# Autodesk Inventor assembly: Tool_Revo
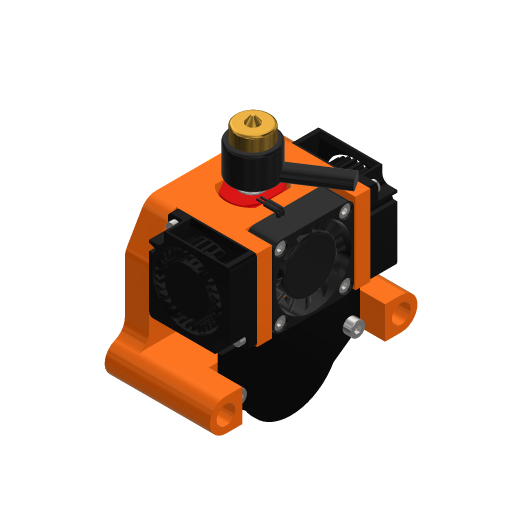
[picture p0: Inventor's stored thumbnail of the model, 512x512]
Saved by Autodesk Inventor 2023.2 (Build 272271000, 271)
## iProperties
Created: 2023-02-09
Part Number: Tool_Revo
Document SubType Name: Assembly
Designer: remop
Author: remop
## Documents named in this file (12)
- C:\Users\remop\OneDrive\Documents\Inventor\3D Printers\LuEVO\Mk5_FullKinematic\Extruders and Tools\Revo Tool\Tool_Revo.iam
- C:\Users\remop\OneDrive\Documents\Inventor\3D Printers\LuEVO\Mk5_FullKinematic\Extruders and Tools\Revo Tool\Tool_Revo.ipt
- C:\Users\remop\OneDrive\Documents\Inventor\3D Printers\LuEVO\Mk5_FullKinematic\XY Motion System\Toolhead\MagToolChanger_CouplerL.ipt
- C:\Users\remop\OneDrive\Documents\Inventor\3D Printers\LuEVO\Mk5_FullKinematic\XY Motion System\Toolhead\MagToolChanger_Magnet.ipt
- C:\Users\remop\OneDrive\Documents\Inventor\3D Printers\LuEVO\Mk5_FullKinematic\Electronics\Mellow Fly SHT36.ipt
- C:\Users\remop\OneDrive\Documents\Inventor\3D Printers\LuEVO\Mk5_FullKinematic\Extruders and Tools\Revo Tool\3010 Blower.ipt
- C:\Users\remop\OneDrive\Documents\Inventor\3D Printers\LuEVO\Mk5_FullKinematic\Extruders and Tools\Revo Tool\3010 Fan.ipt
- C:\Users\remop\OneDrive\Documents\Inventor\3D Printers\LuEVO\Mk5_FullKinematic\Extruders and Tools\Revo Tool\Revo Voron Reference CAD.ipt
- C:\Users\remop\OneDrive\Documents\Inventor\Content Center Files\R2023\en-US\BS EN ISO 4762\BS EN ISO 4762 - M2.5 x 12(1).ipt
- C:\Users\remop\OneDrive\Documents\Inventor\Content Center Files\R2023\en-US\BS EN ISO 4762\BS EN ISO 4762 - M3 x 8(1).ipt
- C:\Users\remop\OneDrive\Documents\Inventor\Content Center Files\R2023\en-US\BS EN ISO 4762\BS EN ISO 4762 - M3 x 12(1).ipt
- C:\Users\remop\OneDrive\Documents\Inventor\Content Center Files\R2023\en-US\BS EN ISO 4762\BS EN ISO 4762 - M2 x 8(1).ipt
## Components (29 placed, 11 different names)
1. Tool_Revo:1 — Mate:1, Mate:2, Mate:3, Mate:4, Mate:5, Mate:6, Mate:7, Mate:8, Mate:9, Rigid:1, Rigid:2, Rigid:3, Rigid:4, Rigid:5, Rigid:6, Flush:2, Mate:15, Mate:16, Flush:3, Mate:17, Flush:7, Flush:8, Mate:20, Rigid:7, Insert:7, Insert:8, Insert:9, Insert:10
2. MagToolChanger_CouplerL:1 — Mate:3, Mate:4, Mate:9
3. MagToolChanger_Magnet:1 — Rigid:1
4. MagToolChanger_CouplerL:2 — Mate:1, Mate:6, Mate:7
5. MagToolChanger_CouplerL:3 — Mate:2, Mate:5, Mate:8
6. MagToolChanger_Magnet:2 — Rigid:2
7. MagToolChanger_Magnet:3 — Rigid:3
8. MagToolChanger_Magnet:4 — Rigid:4
9. MagToolChanger_Magnet:5 — Rigid:5
10. MagToolChanger_Magnet:6 — Rigid:6
11. Mellow Fly SHT36:1 — Flush:7, Flush:8, Mate:20, Insert:5, Insert:6
12. 3010 Blower:1 — Flush:3, Mate:17, Flush:4, Flush:5, Flush:6, Insert:11, Insert:12
13. 3010 Blower:2 — Flush:2, Mate:15, Mate:16, Flush:4, Mate:19, Insert:13, Insert:14
14. 3010 Fan:1 — Flush:5, Mate:19, Flush:6, Insert:1, Insert:2, Insert:3, Insert:4
15. Revo Voron Reference CAD:1 — Rigid:7
16. BS EN ISO 4762 - Metric M2.5 x 12:1 — Insert:1
17. BS EN ISO 4762 - Metric M2.5 x 12:2 — Insert:2
18. BS EN ISO 4762 - Metric M2.5 x 12:3 — Insert:3
19. BS EN ISO 4762 - Metric M2.5 x 12:4 — Insert:4
20. BS EN ISO 4762 - Metric M3 x 8:1 — Insert:5
21. BS EN ISO 4762 - Metric M3 x 8:2 — Insert:6
22. BS EN ISO 4762 - Metric M3 x 12:1 — Insert:7
23. BS EN ISO 4762 - Metric M3 x 12:2 — Insert:8
24. BS EN ISO 4762 - Metric M3 x 12:3 — Insert:9
25. BS EN ISO 4762 - Metric M3 x 12:4 — Insert:10
26. BS EN ISO 4762 - Metric M2 x 8:1 — Insert:11
27. BS EN ISO 4762 - Metric M2 x 8:2 — Insert:12
28. BS EN ISO 4762 - Metric M2 x 8:3 — Insert:13
29. BS EN ISO 4762 - Metric M2 x 8:4 — Insert:14
## Relationships (42: Mate 14, Insert 14, WeldJoint 7, Flush 7)
- Mate:1: Tool_Revo:1 ↔ MagToolChanger_CouplerL:2
- Mate:2: Tool_Revo:1 ↔ MagToolChanger_CouplerL:3
- Mate:3: Tool_Revo:1 ↔ MagToolChanger_CouplerL:1
- Mate:4: Tool_Revo:1 ↔ MagToolChanger_CouplerL:1
- Mate:5: Tool_Revo:1 ↔ MagToolChanger_CouplerL:3
- Mate:6: Tool_Revo:1 ↔ MagToolChanger_CouplerL:2
- Mate:7: Tool_Revo:1 ↔ MagToolChanger_CouplerL:2
- Mate:8: Tool_Revo:1 ↔ MagToolChanger_CouplerL:3
- Mate:9: Tool_Revo:1 ↔ MagToolChanger_CouplerL:1
- Rigid:1 [WeldJoint]: Tool_Revo:1 ↔ MagToolChanger_Magnet:1
- Rigid:2 [WeldJoint]: Tool_Revo:1 ↔ MagToolChanger_Magnet:2
- Rigid:3 [WeldJoint]: Tool_Revo:1 ↔ MagToolChanger_Magnet:3
- Rigid:4 [WeldJoint]: Tool_Revo:1 ↔ MagToolChanger_Magnet:4
- Rigid:5 [WeldJoint]: Tool_Revo:1 ↔ MagToolChanger_Magnet:5
- Rigid:6 [WeldJoint]: Tool_Revo:1 ↔ MagToolChanger_Magnet:6
- Flush:2: Tool_Revo:1 ↔ 3010 Blower:2
- Mate:15: Tool_Revo:1 ↔ 3010 Blower:2
- Mate:16 (10 mm): Tool_Revo:1 ↔ 3010 Blower:2
- Flush:3: Tool_Revo:1 ↔ 3010 Blower:1
- Mate:17: Tool_Revo:1 ↔ 3010 Blower:1
- Flush:4: 3010 Blower:1 ↔ 3010 Blower:2
- Flush:5: 3010 Blower:1 ↔ 3010 Fan:1
- Mate:19 (6 mm): 3010 Blower:2 ↔ 3010 Fan:1
- Flush:6: 3010 Blower:1 ↔ 3010 Fan:1
- Flush:7 (-5.5 mm): Tool_Revo:1 ↔ Mellow Fly SHT36:1
- Flush:8 (5.365 mm): Tool_Revo:1 ↔ Mellow Fly SHT36:1
- Mate:20: Tool_Revo:1 ↔ Mellow Fly SHT36:1
- Rigid:7 [WeldJoint]: Tool_Revo:1 ↔ Revo Voron Reference CAD:1
- Insert:1: 3010 Fan:1 ↔ BS EN ISO 4762 - Metric M2.5 x 12:1
- Insert:2: 3010 Fan:1 ↔ BS EN ISO 4762 - Metric M2.5 x 12:2
- Insert:3: 3010 Fan:1 ↔ BS EN ISO 4762 - Metric M2.5 x 12:3
- Insert:4: 3010 Fan:1 ↔ BS EN ISO 4762 - Metric M2.5 x 12:4
- Insert:5: Mellow Fly SHT36:1 ↔ BS EN ISO 4762 - Metric M3 x 8:1
- Insert:6: Mellow Fly SHT36:1 ↔ BS EN ISO 4762 - Metric M3 x 8:2
- Insert:7: Tool_Revo:1 ↔ BS EN ISO 4762 - Metric M3 x 12:1
- Insert:8: Tool_Revo:1 ↔ BS EN ISO 4762 - Metric M3 x 12:2
- Insert:9: Tool_Revo:1 ↔ BS EN ISO 4762 - Metric M3 x 12:3
- Insert:10: Tool_Revo:1 ↔ BS EN ISO 4762 - Metric M3 x 12:4
- Insert:11: 3010 Blower:1 ↔ BS EN ISO 4762 - Metric M2 x 8:1
- Insert:12: 3010 Blower:1 ↔ BS EN ISO 4762 - Metric M2 x 8:2
- Insert:13: 3010 Blower:2 ↔ BS EN ISO 4762 - Metric M2 x 8:3
- Insert:14: 3010 Blower:2 ↔ BS EN ISO 4762 - Metric M2 x 8:4
